# Autodesk Inventor assembly: Frezowanie_male No.1
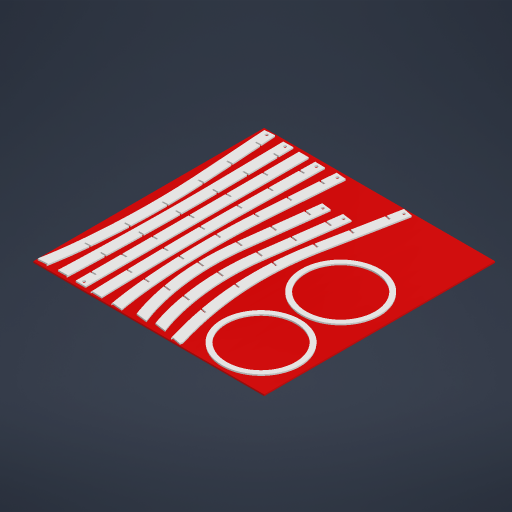
[picture p0: Inventor's stored thumbnail of the model, 512x512]
Saved by Autodesk Inventor 2023 (Build 270158000, 158)
## iProperties
Created: 2023-04-06
Part Number: Frezowanie_male No.1
Document SubType Name: Assembly
Designer: szykr
Author: szykr
## Documents named in this file (12)
- D:\Folder Instalacyjny\GitHub Pliki\Solaris\new model\Frez\Frezowanie_male No.1.iam
- D:\Folder Instalacyjny\GitHub Pliki\Solaris\new model\Frez\Laminat235x235.ipt
- D:\Folder Instalacyjny\GitHub Pliki\Solaris\new model\Frez\Dlugie party(32-47)\Solid33.ipt
- D:\Folder Instalacyjny\GitHub Pliki\Solaris\new model\Frez\Dlugie party(32-47)\Solid35.ipt
- D:\Folder Instalacyjny\GitHub Pliki\Solaris\new model\Frez\Dlugie party(32-47)\Solid37.ipt
- D:\Folder Instalacyjny\GitHub Pliki\Solaris\new model\Frez\Dlugie party(32-47)\Solid39.ipt
- D:\Folder Instalacyjny\GitHub Pliki\Solaris\new model\Frez\Dlugie party(32-47)\Solid41.ipt
- D:\Folder Instalacyjny\GitHub Pliki\Solaris\new model\Frez\Dlugie party(32-47)\Solid43.ipt
- D:\Folder Instalacyjny\GitHub Pliki\Solaris\new model\Frez\Dlugie party(32-47)\Solid45.ipt
- D:\Folder Instalacyjny\GitHub Pliki\Solaris\new model\Frez\Dlugie party(32-47)\Solid47.ipt
- D:\Folder Instalacyjny\GitHub Pliki\Solaris\new model\Frez\Troche Mniejsze(2-31)\Solid6.ipt
- D:\Folder Instalacyjny\GitHub Pliki\Solaris\new model\Frez\Troche Mniejsze(2-31)\Solid16.ipt
## Components (11 placed, 11 different names)
1. Laminat235x235:1 — Angle:1, Mate:1, Angle:2, Mate:2, Angle:3, Mate:3, Mate:4, Mate:5, Mate:6, Mate:7, Mate:8, Mate:9, Mate:10
2. Solid33:1 — Angle:1, Mate:1
3. Solid35:1 — Angle:2, Mate:2
4. Solid37:1 — Angle:3, Mate:3
5. Solid39:1 — Mate:4
6. Solid41:1 — Mate:5
7. Solid43:1 — Mate:6
8. Solid45:1 — Mate:7
9. Solid47:1 — Mate:8
10. Solid6:1 — Mate:9
11. Solid16:1 — Mate:10
## Relationships (13: Mate 10, Angle 3)
- Angle:1 (180 deg): Laminat235x235:1 ↔ Solid33:1
- Mate:1: Laminat235x235:1 ↔ Solid33:1
- Angle:2 (180 deg): Laminat235x235:1 ↔ Solid35:1
- Mate:2: Laminat235x235:1 ↔ Solid35:1
- Angle:3 (180 deg): Laminat235x235:1 ↔ Solid37:1
- Mate:3: Laminat235x235:1 ↔ Solid37:1
- Mate:4: Laminat235x235:1 ↔ Solid39:1
- Mate:5: Laminat235x235:1 ↔ Solid41:1
- Mate:6: Laminat235x235:1 ↔ Solid43:1
- Mate:7: Laminat235x235:1 ↔ Solid45:1
- Mate:8: Laminat235x235:1 ↔ Solid47:1
- Mate:9: Laminat235x235:1 ↔ Solid6:1
- Mate:10: Laminat235x235:1 ↔ Solid16:1
